# Autodesk Inventor assembly: Body
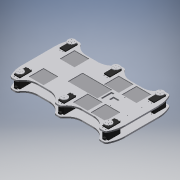
[picture p0: Inventor's stored thumbnail of the model, 180x180]
Saved by Autodesk Inventor 2017 (Build 210142000, 142)
## iProperties
Created: 2017-01-25
Part Number: Body
Document SubType Name: Assembly
Designer: Alexander Miller
Author: Alexander Miller
## Documents named in this file (4)
- D:\Daten\Documents\Git\Hexapod\3DParts\HexPi_v2\Body.iam
- D:\Daten\Documents\Git\Hexapod\3DParts\HexPi_v2\Body_Bottom.ipt
- D:\Daten\Documents\Git\Hexapod\3DParts\HexPi_v2\Serov_with_arm.iam
- D:\Daten\Documents\Git\Hexapod\3DParts\HexPi_v2\Body_Top.ipt
## Components (8 placed, 3 different names)
1. Body_Bottom:1 — Rigid:7
2. Serov_with_arm:1 [sub-assembly] — Rigid:1, Rigid:7
3. Serov_with_arm:2 [sub-assembly] — Rigid:2
4. Serov_with_arm:3 [sub-assembly] — Rigid:3
5. Serov_with_arm:4 [sub-assembly] — Rigid:6
6. Serov_with_arm:5 [sub-assembly] — Rigid:5
7. Serov_with_arm:6 [sub-assembly] — Rigid:4
8. Body_Top:1 — Rigid:1, Rigid:2, Rigid:3, Rigid:4, Rigid:5, Rigid:6
## Relationships (7: WeldJoint 7)
- Rigid:1 [WeldJoint]: Serov_with_arm:1 ↔ Body_Top:1
- Rigid:2 [WeldJoint]: Serov_with_arm:2 ↔ Body_Top:1
- Rigid:3 [WeldJoint]: Serov_with_arm:3 ↔ Body_Top:1
- Rigid:4 [WeldJoint]: Serov_with_arm:6 ↔ Body_Top:1
- Rigid:5 [WeldJoint]: Serov_with_arm:5 ↔ Body_Top:1
- Rigid:6 [WeldJoint]: Serov_with_arm:4 ↔ Body_Top:1
- Rigid:7 [WeldJoint]: Body_Bottom:1 ↔ Serov_with_arm:1
